# Autodesk Inventor assembly: 組合檔
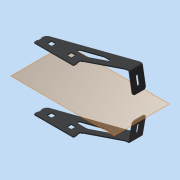
[picture p0: Inventor's stored thumbnail of the model, 180x180]
Saved by Autodesk Inventor 2020 (Build 240168000, 168)
## iProperties
Created: 2015-11-28
Part Number: 組合檔
Document SubType Name: Assembly
Designer: 設計製圖
Author: 設計製圖
## Documents named in this file (3)
- D:\資料庫\設計-3D產品\【May club 】\得利卡-車頂燈架\模型、圖面\吊架-短(R).iam
- D:\資料庫\設計-3D產品\【May club 】\得利卡-車頂燈架\模型、圖面\吊架-短(R).ipt
- D:\資料庫\設計-3D產品\【May club 】\得利卡-車頂燈架\模型、圖面\吊架-短(L)_MIR.ipt
## Components (2 placed, 2 different names)
1. 吊架-短(R):1
2. 吊架-短(L)_MIR:1
## Relationships (1: Flush 1)
- 齊平:1 [Flush] (-100 mm)
